# Autodesk Inventor assembly: s-assy-link1
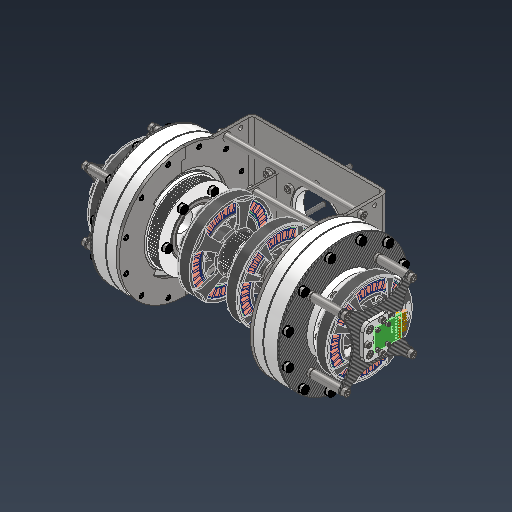
[picture p0: Inventor's stored thumbnail of the model, 512x512]
Saved by Autodesk Inventor 2021 (Build 250183000, 183)
## iProperties
Created: 2021-07-30
Part Number: s-assy-link1
Document SubType Name: Assembly
Designer: yuta0
Mass: 3538.26 g
Surface Area: 7812.66 cm^2
Volume: 1180.98 cm^3
Density: 2.99603 g/cm^3
Author: yuta0
## Documents named in this file (10)
- C:\Users\yuta0\Documents\GitHub\catchrobo_hardware\assy-robot\s-assy-link1.iam
- C:\Users\yuta0\Documents\GitHub\catchrobo_hardware\assy-robot\steel_plate3.ipt
- C:\Users\yuta0\Documents\GitHub\catchrobo_hardware\assy-robot\s-assy-motor-wrist3.iam
- C:\Users\yuta0\Documents\GitHub\catchrobo_hardware\assy-robot\s-assy-unit-j2.iam
- C:\Users\yuta0\Documents\GitHub\catchrobo_hardware\assy-robot\s-assy-unit-j3.iam
- C:\Users\yuta0\Documents\GitHub\catchrobo_hardware\assy-robot\base9.ipt
- C:\Users\yuta0\Documents\GitHub\catchrobo_hardware\assy-robot\CB4-6.ipt
- C:\Users\yuta0\Documents\GitHub\catchrobo_hardware\assy-robot\SFHRW8-75_7-M4-N4_s.ipt
- C:\Users\yuta0\Documents\GitHub\catchrobo_hardware\assy-robot\CB4-35.ipt
- C:\Users\yuta0\Documents\GitHub\catchrobo_hardware\assy-robot\SFHRW8-137-M4-N4_s.ipt
## Components (28 placed, 9 different names)
1. steel_plate3:1 — メイト:7, メイト:8, メイト:9, メイト:10, メイト:11, メイト:12, メイト:13, メイト:14, メイト:15, メイト:16, メイト:17, メイト:18, メイト:38, メイト:39, メイト:40, メイト:41, メイト:42, メイト:55, メイト:56, メイト:57, メイト:58, メイト:59, メイト:60
2. s-assy-motor-wrist3:1 [sub-assembly] — メイト:13, メイト:15, メイト:17, メイト:54
3. s-assy-motor-wrist3:2 [sub-assembly] — メイト:14, メイト:16, メイト:18, メイト:34, メイト:35, メイト:36, メイト:37, メイト:45, メイト:46, メイト:47, メイト:48
4. s-assy-unit-j2:1 [sub-assembly] — メイト:7, メイト:8, メイト:9
5. s-assy-unit-j3:1 [sub-assembly] — メイト:10, メイト:11, メイト:12
6. base9:1 — メイト:38, メイト:39, メイト:40
7. CB4-35:1 — メイト:55, メイト:56
8. CB4-35:2
9. CB4-35:3
10. CB4-35:4
11. CB4-35:5
12. CB4-35:6
13. CB4-6:5 — メイト:41, メイト:42
14. SFHRW8-137-M4-N4_s:1 — メイト:57, メイト:58
15. CB4-6:11 — メイト:59, メイト:60
16. CB4-6:9 — メイト:45, メイト:46
17. CB4-6:10 — メイト:47, メイト:48, メイト:53
18. SFHRW8-75_7-M4-N4_s:1 — メイト:53, メイト:54
19. CB4-6:1 — メイト:34, メイト:35
20. CB4-6:2 — メイト:36, メイト:37
21. CB4-6:12
22. SFHRW8-137-M4-N4_s:2
23. CB4-6:13
24. CB4-6:14
25. CB4-6:15
26. SFHRW8-75_7-M4-N4_s:2
27. CB4-6:16
28. CB4-6:17
## Component patterns: (6 elements, first: CB4-35:1), (2 elements, first: CB4-6:5 + SFHRW8-137-M4-N4_s:1 + CB4-6:11 + CB4-6:9 + CB4-6:10 + SFHRW8-75_7-M4-N4_s:1 + CB4-6:1 + CB4-6:2)
## Relationships (33: Mate 33)
- メイト:7 [Mate]: steel_plate3:1 ↔ s-assy-unit-j2:1
- メイト:8 [Mate]: steel_plate3:1 ↔ s-assy-unit-j2:1
- メイト:9 [Mate]: steel_plate3:1 ↔ s-assy-unit-j2:1
- メイト:10 [Mate]: steel_plate3:1 ↔ s-assy-unit-j3:1
- メイト:11 [Mate]: steel_plate3:1 ↔ s-assy-unit-j3:1
- メイト:12 [Mate]: steel_plate3:1 ↔ s-assy-unit-j3:1
- メイト:13 [Mate]: steel_plate3:1 ↔ s-assy-motor-wrist3:1
- メイト:14 [Mate]: steel_plate3:1 ↔ s-assy-motor-wrist3:2
- メイト:15 [Mate]: steel_plate3:1 ↔ s-assy-motor-wrist3:1
- メイト:16 [Mate]: steel_plate3:1 ↔ s-assy-motor-wrist3:2
- メイト:17 [Mate]: steel_plate3:1 ↔ s-assy-motor-wrist3:1
- メイト:18 [Mate]: steel_plate3:1 ↔ s-assy-motor-wrist3:2
- メイト:34 [Mate]: s-assy-motor-wrist3:2 ↔ CB4-6:1
- メイト:35 [Mate]: s-assy-motor-wrist3:2 ↔ CB4-6:1
- メイト:36 [Mate]: s-assy-motor-wrist3:2 ↔ CB4-6:2
- メイト:37 [Mate]: s-assy-motor-wrist3:2 ↔ CB4-6:2
- メイト:38 [Mate]: steel_plate3:1 ↔ base9:1
- メイト:39 [Mate]: steel_plate3:1 ↔ base9:1
- メイト:40 [Mate]: steel_plate3:1 ↔ base9:1
- メイト:41 [Mate]: steel_plate3:1 ↔ CB4-6:5
- メイト:42 [Mate]: steel_plate3:1 ↔ CB4-6:5
- メイト:45 [Mate]: s-assy-motor-wrist3:2 ↔ CB4-6:9
- メイト:46 [Mate]: s-assy-motor-wrist3:2 ↔ CB4-6:9
- メイト:47 [Mate]: s-assy-motor-wrist3:2 ↔ CB4-6:10
- メイト:48 [Mate]: s-assy-motor-wrist3:2 ↔ CB4-6:10
- メイト:53 [Mate]: CB4-6:10 ↔ SFHRW8-75_7-M4-N4_s:1
- メイト:54 [Mate]: s-assy-motor-wrist3:1 ↔ SFHRW8-75_7-M4-N4_s:1
- メイト:55 [Mate]: steel_plate3:1 ↔ CB4-35:1
- メイト:56 [Mate]: steel_plate3:1 ↔ CB4-35:1
- メイト:57 [Mate]: steel_plate3:1 ↔ SFHRW8-137-M4-N4_s:1
- メイト:58 [Mate]: steel_plate3:1 ↔ SFHRW8-137-M4-N4_s:1
- メイト:59 [Mate]: steel_plate3:1 ↔ CB4-6:11
- メイト:60 [Mate]: steel_plate3:1 ↔ CB4-6:11
